# Autodesk Inventor assembly: cono_assembly
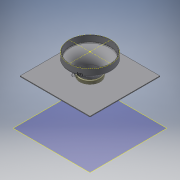
[picture p0: Inventor's stored thumbnail of the model, 180x180]
Saved by Autodesk Inventor 2019 (Build 230136000, 136)
## iProperties
Created: 2019-01-08
Part Number: cono_assembly
Document SubType Name: Assembly
Designer: jmc
Author: jmc
## Documents named in this file (6)
- C:\Users\l0086\Desktop\CatFeeder\cono_assembly.iam
- C:\Users\l0086\Desktop\CatFeeder\cono_nuevo.ipt
- C:\Users\l0086\Desktop\CatFeeder\adaptador_cono.ipt
- C:\Users\l0086\Desktop\CatFeeder\tapa_dummy.ipt
- C:\Users\l0086\Desktop\CatFeeder\trapdoor.ipt
- C:\Users\l0086\Desktop\CatFeeder\cosas\MG995.ipt
## Components (5 placed, 5 different names)
1. cono_nuevo:1
2. adaptador_cono:1 — Flush:1, Flush:2, Flush:3
3. tapa_dummy:1 — Flush:1, Flush:2
4. trapdoor:1 — Flush:3
5. MG995:1
## Relationships (3: Flush 3)
- Flush:1: adaptador_cono:1 ↔ tapa_dummy:1
- Flush:2: adaptador_cono:1 ↔ tapa_dummy:1
- Flush:3: adaptador_cono:1 ↔ trapdoor:1
